# Autodesk Inventor assembly: Assembly_Leg
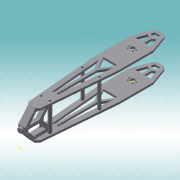
[picture p0: Inventor's stored thumbnail of the model, 180x180]
Saved by Autodesk Inventor 2019 (Build 230136000, 136)
## iProperties
Created: 2019-01-31
Part Number: Assembly_Leg
Document SubType Name: Assembly
Designer: USUARIO
Author: USUARIO
## Documents named in this file (6)
- D:\Users\Documents\Inventor parts\Structure_Charlotte\Structure_Charlotte\Assembly_Leg.iam
- D:\Users\Documents\Inventor parts\Structure_Charlotte\Structure_Charlotte\Leg_part1.ipt
- D:\Users\Documents\Inventor parts\Structure_Charlotte\Structure_Charlotte\Leg_part2.ipt
- D:\Users\Documents\Inventor parts\Structure_Charlotte\Structure_Charlotte\Leg_part3.ipt
- D:\Users\Documents\Inventor parts\Structure_Charlotte\Structure_Charlotte\Standoff.ipt
- D:\Users\Documents\Inventor parts\Structure_Charlotte\Structure_Charlotte\Foot.ipt
## Components (10 placed, 5 different names)
1. Leg_part1:1 — Rigid:1
2. Leg_part2:1 — Rigid:1, Rigid:2, Mate:23, Mate:24, Mate:25, Mate:26, Mate:27, Mate:28, Mate:53, Rigid:3
3. Leg_part1:2 — Rigid:2
4. Leg_part3:1 — Mate:23, Mate:24, Mate:25, Rigid:4, Rigid:5, Rigid:6
5. Leg_part3:2 — Mate:26, Mate:27, Mate:28, Rigid:7
6. Standoff:1 — Rigid:4
7. Standoff:2 — Rigid:5
8. Standoff:3 — Rigid:7
9. Standoff:4 — Rigid:6
10. Foot:1 — Mate:53, Rigid:3
## Relationships (14: WeldJoint 7, Mate 7)
- Rigid:1 [WeldJoint]: Leg_part1:1 ↔ Leg_part2:1
- Rigid:2 [WeldJoint]: Leg_part2:1 ↔ Leg_part1:2
- Mate:23: Leg_part2:1 ↔ Leg_part3:1
- Mate:24: Leg_part2:1 ↔ Leg_part3:1
- Mate:25: Leg_part2:1 ↔ Leg_part3:1
- Mate:26: Leg_part2:1 ↔ Leg_part3:2
- Mate:27: Leg_part2:1 ↔ Leg_part3:2
- Mate:28: Leg_part2:1 ↔ Leg_part3:2
- Mate:53: Leg_part2:1 ↔ Foot:1
- Rigid:3 [WeldJoint]: Leg_part2:1 ↔ Foot:1
- Rigid:4 [WeldJoint]: Leg_part3:1 ↔ Standoff:1
- Rigid:5 [WeldJoint]: Leg_part3:1 ↔ Standoff:2
- Rigid:6 [WeldJoint]: Leg_part3:1 ↔ Standoff:4
- Rigid:7 [WeldJoint]: Leg_part3:2 ↔ Standoff:3
